# Autodesk Inventor assembly: lustro_i_dmd
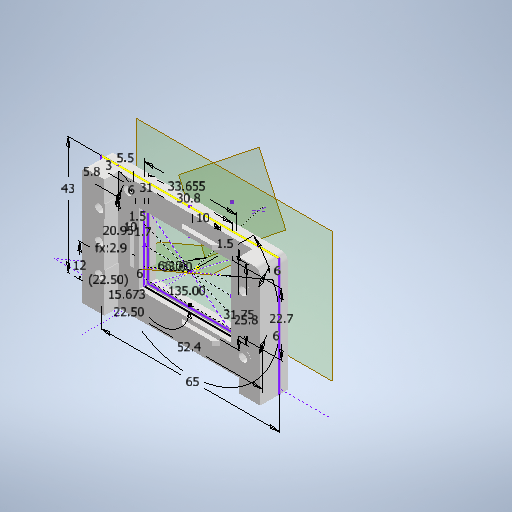
[picture p0: Inventor's stored thumbnail of the model, 512x512]
Saved by Autodesk Inventor 2025.1 (Build 291241020, 241B)
## iProperties
Created: 2024-10-13
Part Number: lustro_i_dmd
Document SubType Name: Assembly
Designer: zychlix
Author: zychlix
## Documents named in this file (3)
- C:\Users\zychlix\Fotolitografia\lustro_i_dmd.iam
- C:\Users\zychlix\Fotolitografia\clamp.ipt
- C:\Users\zychlix\Fotolitografia\lustro.ipt
## Components (2 placed, 2 different names)
1. clamp:1 — Równoległe:1, Równoległe:2, Zestawiające:1, Zestawiające:2
2. lustro:1 — Równoległe:1, Równoległe:2, Zestawiające:1, Zestawiające:2
## Relationships (4: Flush 2, Mate 2)
- Równoległe:1 [Flush]: clamp:1 ↔ lustro:1
- Równoległe:2 [Flush] (13 mm): clamp:1 ↔ lustro:1
- Zestawiające:1 [Mate]: clamp:1 ↔ lustro:1
- Zestawiające:2 [Mate]: clamp:1 ↔ lustro:1
